# Autodesk Inventor assembly: ServerRackSim
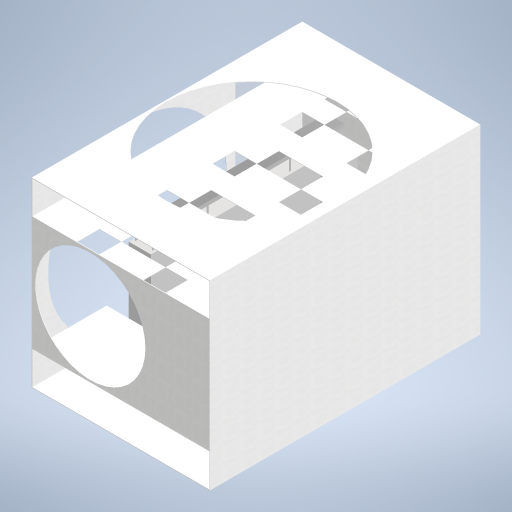
[picture p0: Inventor's stored thumbnail of the model, 512x512]
Saved by Autodesk Inventor 2023.1 (Build 271208000, 208)
## iProperties
Created: 2023-06-06
Part Number: ServerRackSim
Document SubType Name: Assembly
Designer: rwc6
Author: rwc6
## Documents named in this file (6)
- C:\Users\rwc6@nist.gov\Documents\McGarant\ServerRackSim\ServerRackSim.iam
- C:\Users\rwc6@nist.gov\Documents\McGarant\ServerRackSim\ServerRoom.ipt
- C:\Users\rwc6@nist.gov\Documents\McGarant\ServerRackSim\Window.ipt
- C:\Users\rwc6@nist.gov\Documents\McGarant\ServerRackSim\ServerCabinetLeft.ipt
- C:\Users\rwc6@nist.gov\Documents\McGarant\ServerRackSim\ServerCabinetRight.ipt
- C:\Users\rwc6@nist.gov\Documents\McGarant\ServerRackSim\CableTray.ipt
## Components (6 placed, 5 different names)
1. ServerRoom:1 — Mate:1, Angle:1, Mate:3, Angle:2, Mate:4, Angle:3, Mate:7
2. Window:1 — Angle:1, Mate:7
3. ServerCabinetLeft:1 — Mate:3, Angle:2, Mate:5, Angle:4
4. ServerCabinetRight:1 — Mate:4, Angle:3, Mate:6, Angle:5
5. CableTray:1 — Mate:5, Angle:4
6. CableTray:2 — Mate:6, Angle:5
## Relationships (11: Mate 6, Angle 5)
- Mate:1: ServerRoom:1
- Angle:1 (0 deg): ServerRoom:1 ↔ Window:1
- Mate:3: ServerRoom:1 ↔ ServerCabinetLeft:1
- Angle:2 (180 deg): ServerRoom:1 ↔ ServerCabinetLeft:1
- Mate:4: ServerRoom:1 ↔ ServerCabinetRight:1
- Angle:3 (0 deg): ServerRoom:1 ↔ ServerCabinetRight:1
- Mate:5: ServerCabinetLeft:1 ↔ CableTray:1
- Angle:4 (180 deg): ServerCabinetLeft:1 ↔ CableTray:1
- Mate:6: ServerCabinetRight:1 ↔ CableTray:2
- Angle:5 (180 deg): ServerCabinetRight:1 ↔ CableTray:2
- Mate:7: ServerRoom:1 ↔ Window:1
## Named parameters: win_d = 6.4 mm
